# Autodesk Inventor assembly: ForkHandleBar
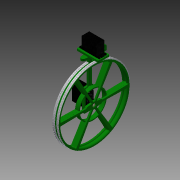
[picture p0: Inventor's stored thumbnail of the model, 180x180]
Saved by Autodesk Inventor 2014 SP1 (Build 180222100, 222)
## iProperties
Created: 2017-01-17
Part Number: ForkHandleBar
Document SubType Name: Assembly
Designer: danielsikar
Author: danielsikar
## Documents named in this file (8)
- C:\Users\danielsikar\Documents\Inventor\IoT-Trike\Assemblies\ForkHandleBar.iam
- C:\Users\danielsikar\Documents\Inventor\IoT-Trike\Parts\TyreR95mm.ipt
- C:\Users\danielsikar\Documents\Inventor\IoT-Trike\Assemblies\ServoAndHorn.iam
- C:\Users\danielsikar\Documents\Inventor\IoT-Trike\STL\Fork2.ipt
- C:\Users\danielsikar\Documents\Inventor\IoT-Trike\Parts\ServoHornPocket2.ipt
- C:\Users\danielsikar\Documents\Inventor\IoT-Trike\STL\ForkSleeve.ipt
- C:\Users\danielsikar\Documents\Inventor\IoT-Trike\STL\TopBar.ipt
- C:\Users\danielsikar\Documents\Inventor\IoT-Trike\Assemblies\DoubleWheelAssy.iam
## Components (9 placed, 7 different names)
1. TyreR95mm:1 — Mate:16, Mate:17, Mate:28
2. ServoAndHorn:1 [sub-assembly] — Flush:1, Flush:7, Mate:24, Mate:25, Mate:26
3. Fork2:1 — Flush:1, Mate:18, Mate:19, Mate:20, Flush:3, Flush:4, Mate:22, Flush:5
4. ServoHornPocket2:2 — Mate:18, Mate:19, Mate:20, Mate:21, Flush:6
5. ForkSleeve:1 — Flush:3, Flush:4
6. ServoAndHorn:2 [sub-assembly] — Mate:21, Mate:22, Mate:23
7. TopBar:1 — Mate:23
8. DoubleWheelAssy:1 [sub-assembly] — Mate:24, Mate:25, Mate:26, Mate:28
9. TyreR95mm:2
## Relationships (20: Mate 13, Flush 7)
- Flush:1: ServoAndHorn:1 ↔ Fork2:1
- Flush:2 (3.25 mm)
- Mate:12
- Mate:16: TyreR95mm:1
- Mate:17: TyreR95mm:1
- Mate:18: Fork2:1 ↔ ServoHornPocket2:2
- Mate:19: Fork2:1 ↔ ServoHornPocket2:2
- Mate:20: Fork2:1 ↔ ServoHornPocket2:2
- Flush:3: Fork2:1 ↔ ForkSleeve:1
- Flush:4: Fork2:1 ↔ ForkSleeve:1
- Mate:21: ServoHornPocket2:2 ↔ ServoAndHorn:2
- Mate:22: Fork2:1 ↔ ServoAndHorn:2
- Flush:5 (30.3 mm): Fork2:1
- Flush:6 (3.4 mm): ServoHornPocket2:2
- Flush:7: ServoAndHorn:1
- Mate:23: ServoAndHorn:2 ↔ TopBar:1
- Mate:24: ServoAndHorn:1 ↔ DoubleWheelAssy:1
- Mate:25: ServoAndHorn:1 ↔ DoubleWheelAssy:1
- Mate:26: ServoAndHorn:1 ↔ DoubleWheelAssy:1
- Mate:28: TyreR95mm:1 ↔ DoubleWheelAssy:1
